# Autodesk Inventor assembly: 300072
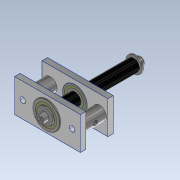
[picture p0: Inventor's stored thumbnail of the model, 180x180]
Saved by Autodesk Inventor 2020 (Build 240168000, 168)
## iProperties
Created: 2021-12-18
Part Number: 300072
Document SubType Name: Assembly
Designer: Byron Robotics
Mass: 236.733 g
Surface Area: 307.265 cm^2
Volume: 58.4435 cm^3
Density: 4.05064 g/cm^3
Author: Byron Robotics
## Documents named in this file (7)
- C:\$WorkingFolder\Projects\2022\Drivebase\300072.iam
- C:\$WorkingFolder\Projects\2022\Drivebase\200289.ipt
- C:\$WorkingFolder\Projects\2022\Drivebase\200287.ipt
- C:\$WorkingFolder\Projects\2022\Drivebase\200288.ipt
- C:\$WorkingFolder\Content Center Files\en-US\en-US\0.5 THUNDER HEX FLANGED BEARING\13.75mm ID x 1.125 OD x 0.313 WD.ipt
- C:\$WorkingFolder\Content Center Files\en-US\en-US\Socket Head Cap Screw - Inch\SHCS - 1_4-20 UNC - 0.375.ipt
- C:\$WorkingFolder\Content Center Files\en-US\en-US\Plain Washer -Inch\ANSI Washer - 1_4 - wide - Type A.ipt
## Components (11 placed, 6 different names)
1. 200289:1 — Mate:8, Mate:9, Mate:10, Mate:11, Mate:14
2. 200289:2 — Mate:12, Mate:13, Mate:14
3. 200287:1 — Mate:1, Flush:1, Mate:2, Mate:3, Angle:1, Mate:16, Mate:17, Mate:18, Mate:21, Mate:22, Mate:23
4. 200288:1 — Mate:5, Mate:6, Mate:9, Mate:11, Symmetry:1, Mate:8
5. 200288:2 — Mate:4, Mate:7, Mate:10, Mate:13, Angle:1, Symmetry:1, Mate:12
6. 0.5 THUNDER HEX FLANGED BEARING 13.75mm ID x 1.125 OD x 0.313 WD:1 — Mate:3, Mate:4, Mate:7
7. 0.5 THUNDER HEX FLANGED BEARING 13.75mm ID x 1.125 OD x 0.313 WD:2 — Mate:2, Mate:5, Mate:6, Mate:20
8. Socket Head Cap Screw - Inch 1/4 - 20 UNC - 3/8:1 — Mate:18, Mate:19
9. Socket Head Cap Screw - Inch 1/4 - 20 UNC - 3/8:2 — Mate:23, Mate:24
10. Plain Washer -Inch 1/4 - wide - Type A:1 — Mate:16, Mate:17, Mate:19, Mate:20
11. Plain Washer -Inch 1/4 - wide - Type A:2 — Mate:21, Mate:22, Mate:24
## Relationships (27: Mate 24, Flush 1, Angle 1, Symmetry 1)
- Mate:1: 200287:1
- Flush:1: 200287:1
- Mate:2: 200287:1 ↔ 0.5 THUNDER HEX FLANGED BEARING 13.75mm ID x 1.125 OD x 0.313 WD:2
- Mate:3: 200287:1 ↔ 0.5 THUNDER HEX FLANGED BEARING 13.75mm ID x 1.125 OD x 0.313 WD:1
- Mate:4: 200288:2 ↔ 0.5 THUNDER HEX FLANGED BEARING 13.75mm ID x 1.125 OD x 0.313 WD:1
- Mate:5: 200288:1 ↔ 0.5 THUNDER HEX FLANGED BEARING 13.75mm ID x 1.125 OD x 0.313 WD:2
- Mate:6: 200288:1 ↔ 0.5 THUNDER HEX FLANGED BEARING 13.75mm ID x 1.125 OD x 0.313 WD:2
- Mate:7: 200288:2 ↔ 0.5 THUNDER HEX FLANGED BEARING 13.75mm ID x 1.125 OD x 0.313 WD:1
- Mate:8: 200289:1 ↔ 200288:1
- Mate:9: 200289:1 ↔ 200288:1
- Mate:10: 200289:1 ↔ 200288:2
- Mate:11: 200289:1 ↔ 200288:1
- Mate:12: 200289:2 ↔ 200288:2
- Mate:13: 200289:2 ↔ 200288:2
- Angle:1 (0 deg): 200287:1 ↔ 200288:2
- Mate:14: 200289:1 ↔ 200289:2
- Symmetry:1: 200288:1 ↔ 200288:2
- Mate:15
- Mate:16: 200287:1 ↔ Plain Washer -Inch 1/4 - wide - Type A:1
- Mate:17: 200287:1 ↔ Plain Washer -Inch 1/4 - wide - Type A:1
- Mate:18: 200287:1 ↔ Socket Head Cap Screw - Inch 1/4 - 20 UNC - 3/8:1
- Mate:19: Socket Head Cap Screw - Inch 1/4 - 20 UNC - 3/8:1 ↔ Plain Washer -Inch 1/4 - wide - Type A:1
- Mate:20: 0.5 THUNDER HEX FLANGED BEARING 13.75mm ID x 1.125 OD x 0.313 WD:2 ↔ Plain Washer -Inch 1/4 - wide - Type A:1
- Mate:21: 200287:1 ↔ Plain Washer -Inch 1/4 - wide - Type A:2
- Mate:22: 200287:1 ↔ Plain Washer -Inch 1/4 - wide - Type A:2
- Mate:23: 200287:1 ↔ Socket Head Cap Screw - Inch 1/4 - 20 UNC - 3/8:2
- Mate:24: Socket Head Cap Screw - Inch 1/4 - 20 UNC - 3/8:2 ↔ Plain Washer -Inch 1/4 - wide - Type A:2
